# Autodesk Inventor assembly: mini sand
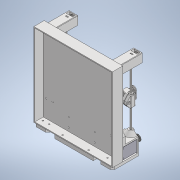
[picture p0: Inventor's stored thumbnail of the model, 180x180]
Saved by Autodesk Inventor 2022 (Build 260153000, 153)
## iProperties
Created: 2022-04-23
Part Number: mini sand
Document SubType Name: Assembly
Designer: Administrator
Title: mini sand v11
Author: Administrator
## Documents named in this file (20)
- Y:\Projects\Mini_Sand_Table\Mini Sand Table.iam
- Y:\Projects\Mini_Sand_Table\4mm x 140mm Rod.ipt
- Y:\Projects\Mini_Sand_Table\4mm x 8mm x 8mm Bushing.ipt
- Y:\Projects\Mini_Sand_Table\roller bearing.ipt
- Y:\Projects\Mini_Sand_Table\4mm x 130mm Rod.ipt
- Y:\Projects\Mini_Sand_Table\GT2 16T Pulley.ipt
- Y:\Projects\Mini_Sand_Table\Magnet Mount.ipt
- Y:\Projects\Mini_Sand_Table\magnet.ipt
- Y:\Projects\Mini_Sand_Table\LM4UU.ipt
- Y:\Projects\Mini_Sand_Table\Table Top.ipt
- Y:\Projects\Mini_Sand_Table\NEMA 11.ipt
- Y:\Projects\Mini_Sand_Table\Belt Retainer.ipt
- Y:\Projects\Mini_Sand_Table\Magnet Mount Lower.ipt
- Y:\Projects\Mini_Sand_Table\SKR PICO.ipt
- Y:\Projects\Mini_Sand_Table\Motor Mount.ipt
- Y:\Projects\Mini_Sand_Table\XY Joiner HSI.iam
- Y:\Projects\Mini_Sand_Table\Idle Bearing Mount HSI.iam
- Y:\Projects\Mini_Sand_Table\M3 Hex Nut.ipt
- Y:\Projects\Mini_Sand_Table\M3 x 10 mm SHCS.ipt
- Y:\Projects\Mini_Sand_Table\Control Board Bracket.ipt
## Components (43 placed, 20 different names)
1. roller bearing:1 — Insert:71, Insert:73
2. roller bearing:2 — Insert:70, Insert:72
3. bushing:5 — Insert:93, Mate:30
4. bushing:6 — Insert:94, Mate:29
5. gt2 pulley 16t v1:1 — Insert:65
6. table mount (1):1 [sub-assembly] — Insert:56, Insert:57, Insert:60, Insert:90
7. roller bearing:3 — Insert:90
8. table mount (1):2 [sub-assembly] — Insert:58, Insert:59, Insert:61, Insert:89
9. roller bearing:4 — Insert:89
10. magnet:1
11. magnet mount:1 — Insert:45, Insert:46, Insert:93, Insert:94
12. XY Joiner HSI:1 [sub-assembly] — Insert:62, Insert:63, Insert:64, Insert:69, Insert:70, Insert:71, Insert:76, Angle:1, Insert:88
13. LM4UU:1 — Insert:63
14. LM4UU:2 — Mate:10, Insert:64
15. LM4UU:3 — Mate:9, Insert:77
16. LM4UU:4 — Insert:78
17. XY Joiner HSI:2 [sub-assembly] — Insert:77, Insert:78, Insert:79, Insert:80, Insert:81, Insert:86, Angle:2, Insert:87
18. 4mm x 140mm Rod:1 — Mate:10, Mate:18, Insert:60
19. 4mm x 140mm Rod:2 — Mate:9, Mate:19, Insert:61
20. Table Top:1 — Mate:15, Mate:20, Mate:21, Mate:22, Insert:56, Insert:57, Insert:58, Insert:59, Mate:23, Mate:25, Mate:26
21. NEMA 11:1 — Insert:66, Insert:67, Insert:68
22. NEMA 11:2 — Insert:54, Insert:55, Insert:65
23. GT2 16T Pulley:2 — Insert:68
24. 4mm x 130mm Rod:2 — Insert:88, Mate:30
25. Belt Retainer:1 — Insert:82, Insert:83, Insert:84, Insert:85
26. Belt Retainer:2 — Insert:72, Insert:73, Insert:74, Insert:75
27. roller bearing:5 — Insert:81, Insert:82
28. roller bearing:6 — Insert:80, Insert:83
29. Magnet Mount Lower:1 — Insert:45, Insert:46
30. 4mm x 130mm Rod:3 — Insert:62, Insert:87, Mate:29
31. SKR PICO:1 — Mate:23, Flush:1, Mate:24, Mate:27, Mate:28, Insert:91, Insert:92
32. Motor Mount:1 — Mate:15, Mate:18, Mate:21, Insert:54, Insert:55, Mate:24
33. Motor Mount:2 — Mate:19, Mate:20, Mate:22, Insert:66, Insert:67, Flush:1
34. M3 Hex Nut:1 — Insert:76, Angle:1
35. M3 x 10 mm SHCS:1 — Insert:75
36. M3 x 10 mm SHCS:2 — Insert:69
37. M3 x 10 mm SHCS:3 — Insert:74
38. M3 x 10 mm SHCS:4 — Insert:84
39. M3 x 10 mm SHCS:5 — Insert:85
40. M3 x 10 mm SHCS:6 — Insert:79
41. M3 Hex Nut:2 — Insert:86, Angle:2
42. Control Board Bracket:1 — Mate:25, Mate:27, Insert:92
43. Control Board Bracket:2 — Mate:26, Mate:28, Insert:91
## Relationships (62: Insert 43, Mate 16, Angle 2, Flush 1)
- Mate:9: LM4UU:3 ↔ 4mm x 140mm Rod:2
- Mate:10: LM4UU:2 ↔ 4mm x 140mm Rod:1
- Insert:45: magnet mount:1 ↔ Magnet Mount Lower:1
- Insert:46: magnet mount:1 ↔ Magnet Mount Lower:1
- Mate:15: Table Top:1 ↔ Motor Mount:1
- Mate:18: 4mm x 140mm Rod:1 ↔ Motor Mount:1
- Mate:19: 4mm x 140mm Rod:2 ↔ Motor Mount:2
- Mate:20: Table Top:1 ↔ Motor Mount:2
- Mate:21: Table Top:1 ↔ Motor Mount:1
- Mate:22: Table Top:1 ↔ Motor Mount:2
- Insert:54: NEMA 11:2 ↔ Motor Mount:1
- Insert:55: NEMA 11:2 ↔ Motor Mount:1
- Insert:56: table mount (1):1 ↔ Table Top:1
- Insert:57: table mount (1):1 ↔ Table Top:1
- Insert:58: table mount (1):2 ↔ Table Top:1
- Insert:59: table mount (1):2 ↔ Table Top:1
- Insert:60: table mount (1):1 ↔ 4mm x 140mm Rod:1
- Insert:61: table mount (1):2 ↔ 4mm x 140mm Rod:2
- Insert:62: XY Joiner HSI:1 ↔ 4mm x 130mm Rod:3
- Insert:63: XY Joiner HSI:1 ↔ LM4UU:1
- Insert:64: XY Joiner HSI:1 ↔ LM4UU:2
- Insert:65: gt2 pulley 16t v1:1 ↔ NEMA 11:2
- Insert:66: NEMA 11:1 ↔ Motor Mount:2
- Insert:67: NEMA 11:1 ↔ Motor Mount:2
- Insert:68: NEMA 11:1 ↔ GT2 16T Pulley:2
- Insert:69: XY Joiner HSI:1 ↔ M3 x 10 mm SHCS:2
- Insert:70: roller bearing:2 ↔ XY Joiner HSI:1
- Insert:71: roller bearing:1 ↔ XY Joiner HSI:1
- Insert:72: roller bearing:2 ↔ Belt Retainer:2
- Insert:73: roller bearing:1 ↔ Belt Retainer:2
- Insert:74: Belt Retainer:2 ↔ M3 x 10 mm SHCS:3
- Insert:75: Belt Retainer:2 ↔ M3 x 10 mm SHCS:1
- Insert:76: XY Joiner HSI:1 ↔ M3 Hex Nut:1
- Angle:1 (0 deg): XY Joiner HSI:1 ↔ M3 Hex Nut:1
- Insert:77: LM4UU:3 ↔ XY Joiner HSI:2
- Insert:78: LM4UU:4 ↔ XY Joiner HSI:2
- Insert:79: XY Joiner HSI:2 ↔ M3 x 10 mm SHCS:6
- Insert:80: XY Joiner HSI:2 ↔ roller bearing:6
- Insert:81: XY Joiner HSI:2 ↔ roller bearing:5
- Insert:82: Belt Retainer:1 ↔ roller bearing:5
- Insert:83: Belt Retainer:1 ↔ roller bearing:6
- Insert:84: Belt Retainer:1 ↔ M3 x 10 mm SHCS:4
- Insert:85: Belt Retainer:1 ↔ M3 x 10 mm SHCS:5
- Insert:86: XY Joiner HSI:2 ↔ M3 Hex Nut:2
- Angle:2 (0 deg): XY Joiner HSI:2 ↔ M3 Hex Nut:2
- Insert:87: XY Joiner HSI:2 ↔ 4mm x 130mm Rod:3
- Insert:88: XY Joiner HSI:1 ↔ 4mm x 130mm Rod:2
- Insert:89: table mount (1):2 ↔ roller bearing:4
- Insert:90: table mount (1):1 ↔ roller bearing:3
- Mate:23: Table Top:1 ↔ SKR PICO:1
- Flush:1: SKR PICO:1 ↔ Motor Mount:2
- Mate:24 (14 mm): SKR PICO:1 ↔ Motor Mount:1
- Mate:25: Table Top:1 ↔ Control Board Bracket:1
- Mate:26: Table Top:1 ↔ Control Board Bracket:2
- Mate:27: SKR PICO:1 ↔ Control Board Bracket:1
- Mate:28: SKR PICO:1 ↔ Control Board Bracket:2
- Insert:91: SKR PICO:1 ↔ Control Board Bracket:2
- Insert:92: SKR PICO:1 ↔ Control Board Bracket:1
- Insert:93 (2 mm): bushing:5 ↔ magnet mount:1
- Insert:94 (2 mm): bushing:6 ↔ magnet mount:1
- Mate:29: bushing:6 ↔ 4mm x 130mm Rod:3
- Mate:30: bushing:5 ↔ 4mm x 130mm Rod:2
